# Autodesk Inventor assembly: Ahmeds_Case_Assembly
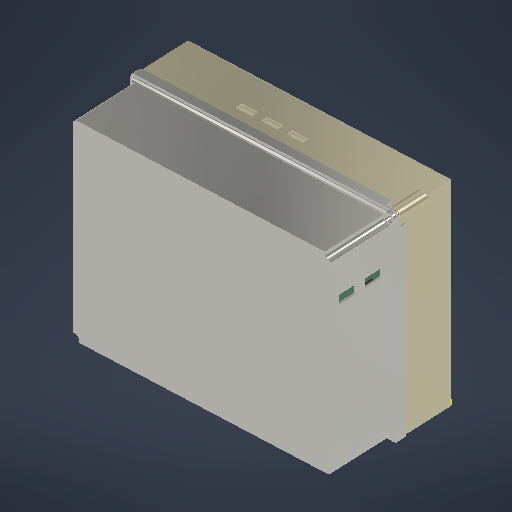
[picture p0: Inventor's stored thumbnail of the model, 512x512]
Saved by Autodesk Inventor 2026.2 (Build 302298000, 298)
## iProperties
Created: 2026-05-13
Part Number: Ahmeds_Case_Assembly
Document SubType Name: Assembly
Designer: Ahmed Youssef
Author: Ahmed Youssef
## Documents named in this file (5)
- C:\Users\Ahmed Youssef\OneDrive\Desktop\Project_Handover\Ahmeds_Enclosure\Ahmeds_Case_Assembly.iam
- C:\Users\Ahmed Youssef\OneDrive\Desktop\ahmed's_SDA1.ipt
- C:\Users\Ahmed Youssef\OneDrive\Desktop\PCB_ZB\PCB_ZB\PCB_ZB.iam
- C:\Users\Ahmed Youssef\OneDrive\Desktop\ahmed's_SDA2.ipt
- C:\Users\Ahmed Youssef\OneDrive\Desktop\LIMIT SWITCH\LIMIT SWITCH\LIMIT SWITCH.ipt
## Components (4 placed, 4 different names)
1. ahmed's_SDA1:1 — Rotational:1, Rotational:3, Rotational:4
2. PCB_ZB:1 [sub-assembly] — Rotational:1
3. ahmed's_SDA2:1 — Rotational:4
4. LIMIT SWITCH:1 — Rotational:3
## Relationships (3: RevoluteJoint 3)
- Rotational:1 [RevoluteJoint]: ahmed's_SDA1:1 ↔ PCB_ZB:1
- Rotational:3 [RevoluteJoint]: ahmed's_SDA1:1 ↔ LIMIT SWITCH:1
- Rotational:4 [RevoluteJoint]: ahmed's_SDA1:1 ↔ ahmed's_SDA2:1
